# Autodesk Inventor assembly: Selection_Shaft Assy
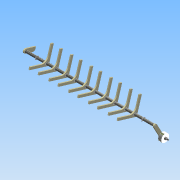
[picture p0: Inventor's stored thumbnail of the model, 180x180]
Saved by Autodesk Inventor 2018.1 (Build 221171000, 171)
## iProperties
Created: 2019-02-14
Part Number: Selection_Shaft Assy
Document SubType Name: Assembly
Designer: James
Author: James
## Documents named in this file (9)
- C:\Users\admin\Desktop\Ball Sorting Machine\Ball-Sorting-Machine\Selection Sort\Selection_Shaft Assy.iam
- C:\Users\admin\Desktop\Ball Sorting Machine\Ball-Sorting-Machine\Selection Sort\Selection_Shaft 1.ipt
- C:\Users\admin\Desktop\Ball Sorting Machine\Ball-Sorting-Machine\Selection Sort\Selection_Selector 1.ipt
- C:\Users\admin\Desktop\Ball Sorting Machine\Ball-Sorting-Machine\Selection Sort\BS 3673 - 6mm External Circlip.ipt
- C:\Users\admin\Desktop\Ball Sorting Machine\Ball-Sorting-Machine\Selection Sort\Selection_Counterweight.ipt
- C:\Users\admin\Desktop\Ball Sorting Machine\Ball-Sorting-Machine\Selection Sort\M3 x 20 - Hex. Head Set Screw (MS).ipt
- C:\Users\admin\Desktop\Ball Sorting Machine\Ball-Sorting-Machine\Selection Sort\Locknut - M3.ipt
- C:\Users\admin\Desktop\Ball Sorting Machine\Ball-Sorting-Machine\Selection Sort\Selection_Weight.ipt
- C:\Users\admin\Desktop\Ball Sorting Machine\Ball-Sorting-Machine\Selection Sort\Selection_Lever 2.ipt
## Components (31 placed, 8 different names)
1. Selection_Shaft 1:1 — Flush:1, Flush:2, Flush:3, Mate:1, Mate:2, Flush:5, Flush:6, Mate:3, Mate:4, Mate:5, Mate:6, Mate:7, Mate:8, Mate:9, Mate:10, Mate:11, Mate:12, Mate:25, Mate:26
2. BS 3673 - 6mm External Circlip:11 — Mate:7, Mate:8, Flush:8
3. BS 3673 - 6mm External Circlip:12 — Mate:9, Mate:10, Flush:7, Flush:8
4. Selection_Counterweight:1 — Mate:11, Angle:1, Mate:12, Mate:13, Mate:14, Mate:17
5. Hex. Head Set Screw (MS) - M3 x 10:1 — Mate:13, Mate:14, Mate:15, Mate:16, Mate:22, Mate:23, Mate:24
6. Locknut - M3:1 — Mate:15, Mate:21
7. Selection_Weight:1 — Mate:16, Mate:17, Mate:18
8. Selection_Weight:2 — Mate:18, Mate:19, Mate:24
9. Selection_Weight:3 — Mate:19, Mate:20, Mate:23
10. Selection_Weight:4 — Mate:20, Mate:21, Mate:22
11. Selection_Lever 2:1 — Mate:25, Mate:26, Angle:2
12. BS 3673 - 6mm External Circlip:2 — Mate:4, Mate:5, Flush:7, Flush:9
13. Selection_Selector 1:1 — Mate:2, Flush:4, Flush:5, Angle:1
14. BS 3673 - 6mm External Circlip:1 — Mate:3, Mate:6, Flush:9
15. Selection_Selector 1:2 — Mate:1, Flush:4, Flush:6
16. BS 3673 - 6mm External Circlip:3
17. Selection_Selector 1:3
18. BS 3673 - 6mm External Circlip:4
19. Selection_Selector 1:4
20. BS 3673 - 6mm External Circlip:5
21. Selection_Selector 1:5
22. BS 3673 - 6mm External Circlip:6
23. Selection_Selector 1:6
24. BS 3673 - 6mm External Circlip:7
25. Selection_Selector 1:7
26. BS 3673 - 6mm External Circlip:8
27. Selection_Selector 1:8
28. BS 3673 - 6mm External Circlip:9
29. Selection_Selector 1:9
30. BS 3673 - 6mm External Circlip:10
31. Selection_Selector 1:10 — Angle:2
## Component patterns: (5 elements, first: BS 3673 - 6mm External Circlip:2 + Selection_Selector 1:1 + BS 3673 - 6mm External Circlip:1 + Selection_Selector 1:2)
## Relationships (37: Mate 26, Flush 9, Angle 2)
- Flush:1: Selection_Shaft 1:1
- Flush:2: Selection_Shaft 1:1
- Flush:3: Selection_Shaft 1:1
- Mate:1: Selection_Shaft 1:1 ↔ Selection_Selector 1:2
- Mate:2: Selection_Shaft 1:1 ↔ Selection_Selector 1:1
- Flush:4: Selection_Selector 1:1 ↔ Selection_Selector 1:2
- Flush:5: Selection_Shaft 1:1 ↔ Selection_Selector 1:1
- Flush:6: Selection_Shaft 1:1 ↔ Selection_Selector 1:2
- Mate:3: Selection_Shaft 1:1 ↔ BS 3673 - 6mm External Circlip:1
- Mate:4: Selection_Shaft 1:1 ↔ BS 3673 - 6mm External Circlip:2
- Mate:5: Selection_Shaft 1:1 ↔ BS 3673 - 6mm External Circlip:2
- Mate:6: Selection_Shaft 1:1 ↔ BS 3673 - 6mm External Circlip:1
- Mate:7: Selection_Shaft 1:1 ↔ BS 3673 - 6mm External Circlip:11
- Mate:8: Selection_Shaft 1:1 ↔ BS 3673 - 6mm External Circlip:11
- Mate:9: Selection_Shaft 1:1 ↔ BS 3673 - 6mm External Circlip:12
- Mate:10: Selection_Shaft 1:1 ↔ BS 3673 - 6mm External Circlip:12
- Flush:7: BS 3673 - 6mm External Circlip:12 ↔ BS 3673 - 6mm External Circlip:2
- Flush:8: BS 3673 - 6mm External Circlip:11 ↔ BS 3673 - 6mm External Circlip:12
- Mate:11: Selection_Shaft 1:1 ↔ Selection_Counterweight:1
- Angle:1 (45 deg): Selection_Counterweight:1 ↔ Selection_Selector 1:1
- Mate:12: Selection_Shaft 1:1 ↔ Selection_Counterweight:1
- Flush:9: BS 3673 - 6mm External Circlip:2 ↔ BS 3673 - 6mm External Circlip:1
- Mate:13: Selection_Counterweight:1 ↔ Hex. Head Set Screw (MS) - M3 x 10:1
- Mate:14: Selection_Counterweight:1 ↔ Hex. Head Set Screw (MS) - M3 x 10:1
- Mate:15: Hex. Head Set Screw (MS) - M3 x 10:1 ↔ Locknut - M3:1
- Mate:16: Hex. Head Set Screw (MS) - M3 x 10:1 ↔ Selection_Weight:1
- Mate:17: Selection_Counterweight:1 ↔ Selection_Weight:1
- Mate:18: Selection_Weight:1 ↔ Selection_Weight:2
- Mate:19: Selection_Weight:2 ↔ Selection_Weight:3
- Mate:20: Selection_Weight:3 ↔ Selection_Weight:4
- Mate:21: Locknut - M3:1 ↔ Selection_Weight:4
- Mate:22: Hex. Head Set Screw (MS) - M3 x 10:1 ↔ Selection_Weight:4
- Mate:23: Hex. Head Set Screw (MS) - M3 x 10:1 ↔ Selection_Weight:3
- Mate:24: Hex. Head Set Screw (MS) - M3 x 10:1 ↔ Selection_Weight:2
- Mate:25: Selection_Shaft 1:1 ↔ Selection_Lever 2:1
- Mate:26: Selection_Shaft 1:1 ↔ Selection_Lever 2:1
- Angle:2 (0 deg): Selection_Lever 2:1 ↔ Selection_Selector 1:10
